# Autodesk Inventor assembly: baseRoulante
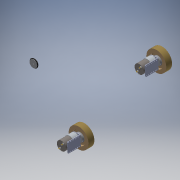
[picture p0: Inventor's stored thumbnail of the model, 180x180]
Saved by Autodesk Inventor 2017 (Build 210142000, 142)
## iProperties
Created: 2017-12-17
Part Number: baseRoulante
Document SubType Name: Assembly
Designer: franc
Author: franc
## Documents named in this file (6)
- C:\Users\franc\Desktop\EsialRobotik\Mecanique\base_roulante\composants\baseRoulante.iam
- C:\Users\franc\Desktop\EsialRobotik\Mecanique\base_roulante\composants\37d-gearmotor-19-30.ipt
- C:\Users\franc\Desktop\EsialRobotik\Mecanique\base_roulante\composants\support_moteur.ipt
- C:\Users\franc\Desktop\EsialRobotik\Mecanique\base_roulante\composants\moyeu_serrage_conique.ipt
- C:\Users\franc\Desktop\EsialRobotik\Mecanique\base_roulante\composants\Colson_Wheel_3in_x_7_8in.ipt
- C:\Users\franc\Desktop\EsialRobotik\Mecanique\base_roulante\composants\Roue de mesure Scancon 100 mm -ID64.ipt
## Components (9 placed, 5 different names)
1. 37d-gearmotor-19-30:1 — Placage:2, Placage:3, Placage:5, Placage:6, Placage:8
2. support_moteur:1 — Placage:2, Placage:3, Placage:8
3. moyeu_serrage_conique:1 — Placage:5, Placage:6, Placage:7, Affleurement:1
4. Colson_Wheel_3in_x_7_8in:1 — Placage:7, Affleurement:1
5. 37d-gearmotor-19-30:2
6. support_moteur:2
7. moyeu_serrage_conique:2
8. Colson_Wheel_3in_x_7_8in:2
9. Roue de mesure Scancon 100 mm -ID64:1
## Relationships (14: Mate 12, Flush 2)
- Placage:2 [Mate]: 37d-gearmotor-19-30:1 ↔ support_moteur:1
- Placage:3 [Mate]: 37d-gearmotor-19-30:1 ↔ support_moteur:1
- Placage:5 [Mate]: 37d-gearmotor-19-30:1 ↔ moyeu_serrage_conique:1
- Placage:6 [Mate]: 37d-gearmotor-19-30:1 ↔ moyeu_serrage_conique:1
- Placage:7 [Mate]: moyeu_serrage_conique:1 ↔ Colson_Wheel_3in_x_7_8in:1
- Affleurement:1 [Flush]: moyeu_serrage_conique:1 ↔ Colson_Wheel_3in_x_7_8in:1
- Placage:8 [Mate]: 37d-gearmotor-19-30:1 ↔ support_moteur:1
- [Mate]: 37d-gearmotor-19-30:2 ↔ support_moteur:2
- [Mate]: 37d-gearmotor-19-30:2 ↔ support_moteur:2
- [Mate]: 37d-gearmotor-19-30:2 ↔ moyeu_serrage_conique:2
- [Mate]: 37d-gearmotor-19-30:2 ↔ moyeu_serrage_conique:2
- [Mate]: moyeu_serrage_conique:2 ↔ Colson_Wheel_3in_x_7_8in:2
- [Flush]: moyeu_serrage_conique:2 ↔ Colson_Wheel_3in_x_7_8in:2
- [Mate]: 37d-gearmotor-19-30:2 ↔ support_moteur:2
## Named parameters: d15_d4 = 0 mm, d16_d9 = 0 mm, d17_d11 = 0 mm, d18_d12 = 0 mm, d19_d13 = 0 mm, d20_d14 = 0 mm, d21_d1 = 0 mm
